# Autodesk Inventor assembly: BG_Mattenwagen
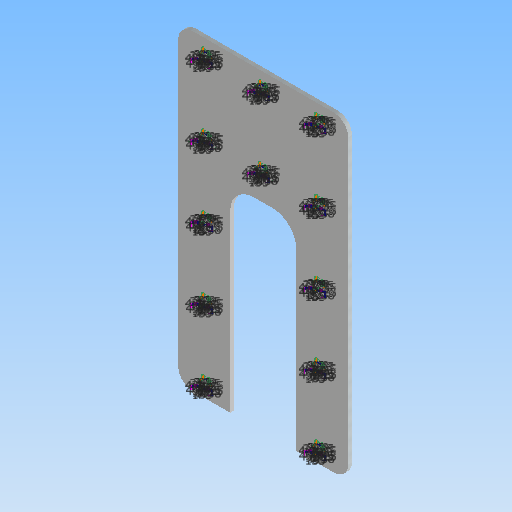
[picture p0: Inventor's stored thumbnail of the model, 512x512]
Saved by Autodesk Inventor 2024.4 (Build 284460000, 460)
## iProperties
Created: 2026-01-22
Part Number: BG_Mattenwagen
Document SubType Name: Assembly
Designer: windows-desktop
Mass: 56051.1 g
Surface Area: 201169 cm^2
Volume: 54823 cm^3
Density: 1.0224 g/cm^3
Author: windows-desktop
## Documents named in this file (4)
- C:\Users\windows-desktop\Desktop\Studium\Konstruktion\VaultWorkspace\Daten\I60-Konstruktion\I60-Gruppe-4\Bluhm\Daten\I60-Konstruktion\I60-Gruppe-4\Bluhm\Transport\BG_Mattenwagen.iam
- C:\Users\windows-desktop\Desktop\Studium\Konstruktion\VaultWorkspace\Daten\I60-Konstruktion\I60-Gruppe-4\Bluhm\Daten\I60-Konstruktion\I60-Gruppe-4\Bluhm\Transport\Wagen_Platte.ipt
- C:\Users\windows-desktop\Desktop\Studium\Konstruktion\VaultWorkspace\Daten\I60-Konstruktion\I60-Gruppe-4\Bluhm\Daten\I60-Konstruktion\I60-Gruppe-4\Bluhm\Transport\BG_Rolle.iam
- C:\Users\windows-desktop\Desktop\Studium\Konstruktion\VaultWorkspace\Daten\I60-Konstruktion\I60-Gruppe-4\Bluhm\Normteile\de-DE\ISO 4762(1)\DIN EN ISO 4762 - M10 x 16.ipt
## Components (61 placed, 3 different names)
1. Wagen_Platte:1 — Einfügen:1, Einfügen:2, Einfügen:3, Einfügen:4, Einfügen:5, Einfügen:6, Passend:1, Passend:3, Passend:5, Passend:7, Passend:9, Passend:11, Passend:13, Passend:15, Passend:17, Passend:19, Passend:21, Passend:23, Passend:25, Passend:27, Passend:29, Passend:31, Passend:33, Passend:35, Passend:37, Passend:39, Passend:41, Passend:43, Passend:45, Passend:47, Passend:49, Passend:51, Passend:53, Passend:55, Passend:57, Passend:59, Passend:61, Passend:63, Passend:65, Passend:67, Passend:69, Passend:71, Passend:73, Passend:75, Passend:77, Passend:79, Passend:81, Passend:83, Passend:85, Passend:87, Passend:89, Passend:91, Passend:93, Passend:95
2. DIN EN ISO 4762 M10 x 16:1 — Passend:1, Passend:2
3. DIN EN ISO 4762 M10 x 16:2 — Passend:3, Passend:4
4. DIN EN ISO 4762 M10 x 16:3 — Passend:5, Passend:6
5. DIN EN ISO 4762 M10 x 16:4 — Passend:7, Passend:8
6. DIN EN ISO 4762 M10 x 16:5 — Passend:9, Passend:10
7. DIN EN ISO 4762 M10 x 16:6 — Passend:11, Passend:12
8. DIN EN ISO 4762 M10 x 16:7 — Passend:13, Passend:14
9. DIN EN ISO 4762 M10 x 16:8 — Passend:15, Passend:16
10. DIN EN ISO 4762 M10 x 16:9 — Passend:17, Passend:18
11. DIN EN ISO 4762 M10 x 16:10 — Passend:19, Passend:20
12. DIN EN ISO 4762 M10 x 16:11 — Passend:21, Passend:22
13. DIN EN ISO 4762 M10 x 16:12 — Passend:23, Passend:24
14. DIN EN ISO 4762 M10 x 16:13 — Passend:25, Passend:26
15. DIN EN ISO 4762 M10 x 16:14 — Passend:27, Passend:28
16. DIN EN ISO 4762 M10 x 16:15 — Passend:29, Passend:30
17. DIN EN ISO 4762 M10 x 16:16 — Passend:31, Passend:32
18. DIN EN ISO 4762 M10 x 16:17 — Passend:33, Passend:34
19. DIN EN ISO 4762 M10 x 16:18 — Passend:35, Passend:36
20. DIN EN ISO 4762 M10 x 16:19 — Passend:37, Passend:38
21. DIN EN ISO 4762 M10 x 16:20 — Passend:39, Passend:40
22. DIN EN ISO 4762 M10 x 16:21 — Passend:41, Passend:42
23. DIN EN ISO 4762 M10 x 16:22 — Passend:43, Passend:44
24. DIN EN ISO 4762 M10 x 16:23 — Passend:45, Passend:46
25. DIN EN ISO 4762 M10 x 16:24 — Passend:47, Passend:48
26. DIN EN ISO 4762 M10 x 16:25 — Passend:49, Passend:50
27. DIN EN ISO 4762 M10 x 16:26 — Passend:51, Passend:52
28. DIN EN ISO 4762 M10 x 16:27 — Passend:53, Passend:54
29. DIN EN ISO 4762 M10 x 16:28 — Passend:55, Passend:56
30. DIN EN ISO 4762 M10 x 16:29 — Passend:57, Passend:58
31. DIN EN ISO 4762 M10 x 16:30 — Passend:59, Passend:60
32. DIN EN ISO 4762 M10 x 16:31 — Passend:61, Passend:62
33. DIN EN ISO 4762 M10 x 16:32 — Passend:63, Passend:64
34. DIN EN ISO 4762 M10 x 16:33 — Passend:65, Passend:66
35. DIN EN ISO 4762 M10 x 16:34 — Passend:67, Passend:68
36. DIN EN ISO 4762 M10 x 16:35 — Passend:69, Passend:70
37. DIN EN ISO 4762 M10 x 16:36 — Passend:71, Passend:72
38. DIN EN ISO 4762 M10 x 16:37 — Passend:73, Passend:74
39. DIN EN ISO 4762 M10 x 16:38 — Passend:75, Passend:76
40. DIN EN ISO 4762 M10 x 16:39 — Passend:77, Passend:78
41. DIN EN ISO 4762 M10 x 16:40 — Passend:79, Passend:80
42. DIN EN ISO 4762 M10 x 16:41 — Passend:81, Passend:82
43. DIN EN ISO 4762 M10 x 16:42 — Passend:83, Passend:84
44. DIN EN ISO 4762 M10 x 16:43 — Passend:85, Passend:86
45. DIN EN ISO 4762 M10 x 16:44 — Passend:87, Passend:88
46. DIN EN ISO 4762 M10 x 16:45 — Passend:89, Passend:90
47. DIN EN ISO 4762 M10 x 16:46 — Passend:91, Passend:92
48. DIN EN ISO 4762 M10 x 16:47 — Passend:93, Passend:94
49. DIN EN ISO 4762 M10 x 16:48 — Passend:95, Passend:96
50. BG_Rolle:3 [sub-assembly] — Einfügen:1, Einfügen:2
51. BG_Rolle:4 [sub-assembly]
52. BG_Rolle:5 [sub-assembly]
53. BG_Rolle:6 [sub-assembly]
54. BG_Rolle:7 [sub-assembly]
55. BG_Rolle:1 [sub-assembly] — Einfügen:3, Einfügen:4
56. BG_Rolle:8 [sub-assembly]
57. BG_Rolle:9 [sub-assembly] — Einfügen:5, Einfügen:6
58. BG_Rolle:10 [sub-assembly]
59. BG_Rolle:11 [sub-assembly]
60. BG_Rolle:12 [sub-assembly] — Passend:2, Passend:4, Passend:6, Passend:8, Passend:10, Passend:12, Passend:14, Passend:16, Passend:18, Passend:20, Passend:22, Passend:24, Passend:26, Passend:28, Passend:30, Passend:32, Passend:34, Passend:36, Passend:38, Passend:40, Passend:42, Passend:44, Passend:46, Passend:48, Passend:50, Passend:52, Passend:54, Passend:56, Passend:58, Passend:60, Passend:62, Passend:64, Passend:66, Passend:68, Passend:70, Passend:72, Passend:74, Passend:76, Passend:78, Passend:80, Passend:82, Passend:84, Passend:86, Passend:88, Passend:90, Passend:92, Passend:94, Passend:96
61. BG_Rolle:13 [sub-assembly]
## Component patterns: (5 elements, first: BG_Rolle:3), (2 elements, first: BG_Rolle:1), (5 elements, first: BG_Rolle:9)
## Relationships (102: Mate 96, Insert 6)
- Einfügen:1 [Insert]: Wagen_Platte:1 ↔ BG_Rolle:3
- Einfügen:2 [Insert]: Wagen_Platte:1 ↔ BG_Rolle:3
- Einfügen:3 [Insert]: Wagen_Platte:1 ↔ BG_Rolle:1
- Einfügen:4 [Insert]: Wagen_Platte:1 ↔ BG_Rolle:1
- Einfügen:5 [Insert]: Wagen_Platte:1 ↔ BG_Rolle:9
- Einfügen:6 [Insert]: Wagen_Platte:1 ↔ BG_Rolle:9
- Passend:1 [Mate]: Wagen_Platte:1 ↔ DIN EN ISO 4762 M10 x 16:1
- Passend:2 [Mate]: DIN EN ISO 4762 M10 x 16:1 ↔ BG_Rolle:12
- Passend:3 [Mate]: Wagen_Platte:1 ↔ DIN EN ISO 4762 M10 x 16:2
- Passend:4 [Mate]: DIN EN ISO 4762 M10 x 16:2 ↔ BG_Rolle:12
- Passend:5 [Mate]: Wagen_Platte:1 ↔ DIN EN ISO 4762 M10 x 16:3
- Passend:6 [Mate]: DIN EN ISO 4762 M10 x 16:3 ↔ BG_Rolle:12
- Passend:7 [Mate]: Wagen_Platte:1 ↔ DIN EN ISO 4762 M10 x 16:4
- Passend:8 [Mate]: DIN EN ISO 4762 M10 x 16:4 ↔ BG_Rolle:12
- Passend:9 [Mate]: Wagen_Platte:1 ↔ DIN EN ISO 4762 M10 x 16:5
- Passend:10 [Mate]: DIN EN ISO 4762 M10 x 16:5 ↔ BG_Rolle:12
- Passend:11 [Mate]: Wagen_Platte:1 ↔ DIN EN ISO 4762 M10 x 16:6
- Passend:12 [Mate]: DIN EN ISO 4762 M10 x 16:6 ↔ BG_Rolle:12
- Passend:13 [Mate]: Wagen_Platte:1 ↔ DIN EN ISO 4762 M10 x 16:7
- Passend:14 [Mate]: DIN EN ISO 4762 M10 x 16:7 ↔ BG_Rolle:12
- Passend:15 [Mate]: Wagen_Platte:1 ↔ DIN EN ISO 4762 M10 x 16:8
- Passend:16 [Mate]: DIN EN ISO 4762 M10 x 16:8 ↔ BG_Rolle:12
- Passend:17 [Mate]: Wagen_Platte:1 ↔ DIN EN ISO 4762 M10 x 16:9
- Passend:18 [Mate]: DIN EN ISO 4762 M10 x 16:9 ↔ BG_Rolle:12
- Passend:19 [Mate]: Wagen_Platte:1 ↔ DIN EN ISO 4762 M10 x 16:10
- Passend:20 [Mate]: DIN EN ISO 4762 M10 x 16:10 ↔ BG_Rolle:12
- Passend:21 [Mate]: Wagen_Platte:1 ↔ DIN EN ISO 4762 M10 x 16:11
- Passend:22 [Mate]: DIN EN ISO 4762 M10 x 16:11 ↔ BG_Rolle:12
- Passend:23 [Mate]: Wagen_Platte:1 ↔ DIN EN ISO 4762 M10 x 16:12
- Passend:24 [Mate]: DIN EN ISO 4762 M10 x 16:12 ↔ BG_Rolle:12
- Passend:25 [Mate]: Wagen_Platte:1 ↔ DIN EN ISO 4762 M10 x 16:13
- Passend:26 [Mate]: DIN EN ISO 4762 M10 x 16:13 ↔ BG_Rolle:12
- Passend:27 [Mate]: Wagen_Platte:1 ↔ DIN EN ISO 4762 M10 x 16:14
- Passend:28 [Mate]: DIN EN ISO 4762 M10 x 16:14 ↔ BG_Rolle:12
- Passend:29 [Mate]: Wagen_Platte:1 ↔ DIN EN ISO 4762 M10 x 16:15
- Passend:30 [Mate]: DIN EN ISO 4762 M10 x 16:15 ↔ BG_Rolle:12
- Passend:31 [Mate]: Wagen_Platte:1 ↔ DIN EN ISO 4762 M10 x 16:16
- Passend:32 [Mate]: DIN EN ISO 4762 M10 x 16:16 ↔ BG_Rolle:12
- Passend:33 [Mate]: Wagen_Platte:1 ↔ DIN EN ISO 4762 M10 x 16:17
- Passend:34 [Mate]: DIN EN ISO 4762 M10 x 16:17 ↔ BG_Rolle:12
- Passend:35 [Mate]: Wagen_Platte:1 ↔ DIN EN ISO 4762 M10 x 16:18
- Passend:36 [Mate]: DIN EN ISO 4762 M10 x 16:18 ↔ BG_Rolle:12
- Passend:37 [Mate]: Wagen_Platte:1 ↔ DIN EN ISO 4762 M10 x 16:19
- Passend:38 [Mate]: DIN EN ISO 4762 M10 x 16:19 ↔ BG_Rolle:12
- Passend:39 [Mate]: Wagen_Platte:1 ↔ DIN EN ISO 4762 M10 x 16:20
- Passend:40 [Mate]: DIN EN ISO 4762 M10 x 16:20 ↔ BG_Rolle:12
- Passend:41 [Mate]: Wagen_Platte:1 ↔ DIN EN ISO 4762 M10 x 16:21
- Passend:42 [Mate]: DIN EN ISO 4762 M10 x 16:21 ↔ BG_Rolle:12
- Passend:43 [Mate]: Wagen_Platte:1 ↔ DIN EN ISO 4762 M10 x 16:22
- Passend:44 [Mate]: DIN EN ISO 4762 M10 x 16:22 ↔ BG_Rolle:12
- Passend:45 [Mate]: Wagen_Platte:1 ↔ DIN EN ISO 4762 M10 x 16:23
- Passend:46 [Mate]: DIN EN ISO 4762 M10 x 16:23 ↔ BG_Rolle:12
- Passend:47 [Mate]: Wagen_Platte:1 ↔ DIN EN ISO 4762 M10 x 16:24
- Passend:48 [Mate]: DIN EN ISO 4762 M10 x 16:24 ↔ BG_Rolle:12
- Passend:49 [Mate]: Wagen_Platte:1 ↔ DIN EN ISO 4762 M10 x 16:25
- Passend:50 [Mate]: DIN EN ISO 4762 M10 x 16:25 ↔ BG_Rolle:12
- Passend:51 [Mate]: Wagen_Platte:1 ↔ DIN EN ISO 4762 M10 x 16:26
- Passend:52 [Mate]: DIN EN ISO 4762 M10 x 16:26 ↔ BG_Rolle:12
- Passend:53 [Mate]: Wagen_Platte:1 ↔ DIN EN ISO 4762 M10 x 16:27
- Passend:54 [Mate]: DIN EN ISO 4762 M10 x 16:27 ↔ BG_Rolle:12
- Passend:55 [Mate]: Wagen_Platte:1 ↔ DIN EN ISO 4762 M10 x 16:28
- Passend:56 [Mate]: DIN EN ISO 4762 M10 x 16:28 ↔ BG_Rolle:12
- Passend:57 [Mate]: Wagen_Platte:1 ↔ DIN EN ISO 4762 M10 x 16:29
- Passend:58 [Mate]: DIN EN ISO 4762 M10 x 16:29 ↔ BG_Rolle:12
- Passend:59 [Mate]: Wagen_Platte:1 ↔ DIN EN ISO 4762 M10 x 16:30
- Passend:60 [Mate]: DIN EN ISO 4762 M10 x 16:30 ↔ BG_Rolle:12
- Passend:61 [Mate]: Wagen_Platte:1 ↔ DIN EN ISO 4762 M10 x 16:31
- Passend:62 [Mate]: DIN EN ISO 4762 M10 x 16:31 ↔ BG_Rolle:12
- Passend:63 [Mate]: Wagen_Platte:1 ↔ DIN EN ISO 4762 M10 x 16:32
- Passend:64 [Mate]: DIN EN ISO 4762 M10 x 16:32 ↔ BG_Rolle:12
- Passend:65 [Mate]: Wagen_Platte:1 ↔ DIN EN ISO 4762 M10 x 16:33
- Passend:66 [Mate]: DIN EN ISO 4762 M10 x 16:33 ↔ BG_Rolle:12
- Passend:67 [Mate]: Wagen_Platte:1 ↔ DIN EN ISO 4762 M10 x 16:34
- Passend:68 [Mate]: DIN EN ISO 4762 M10 x 16:34 ↔ BG_Rolle:12
- Passend:69 [Mate]: Wagen_Platte:1 ↔ DIN EN ISO 4762 M10 x 16:35
- Passend:70 [Mate]: DIN EN ISO 4762 M10 x 16:35 ↔ BG_Rolle:12
- Passend:71 [Mate]: Wagen_Platte:1 ↔ DIN EN ISO 4762 M10 x 16:36
- Passend:72 [Mate]: DIN EN ISO 4762 M10 x 16:36 ↔ BG_Rolle:12
- Passend:73 [Mate]: Wagen_Platte:1 ↔ DIN EN ISO 4762 M10 x 16:37
- Passend:74 [Mate]: DIN EN ISO 4762 M10 x 16:37 ↔ BG_Rolle:12
- Passend:75 [Mate]: Wagen_Platte:1 ↔ DIN EN ISO 4762 M10 x 16:38
- Passend:76 [Mate]: DIN EN ISO 4762 M10 x 16:38 ↔ BG_Rolle:12
- Passend:77 [Mate]: Wagen_Platte:1 ↔ DIN EN ISO 4762 M10 x 16:39
- Passend:78 [Mate]: DIN EN ISO 4762 M10 x 16:39 ↔ BG_Rolle:12
- Passend:79 [Mate]: Wagen_Platte:1 ↔ DIN EN ISO 4762 M10 x 16:40
- Passend:80 [Mate]: DIN EN ISO 4762 M10 x 16:40 ↔ BG_Rolle:12
- Passend:81 [Mate]: Wagen_Platte:1 ↔ DIN EN ISO 4762 M10 x 16:41
- Passend:82 [Mate]: DIN EN ISO 4762 M10 x 16:41 ↔ BG_Rolle:12
- Passend:83 [Mate]: Wagen_Platte:1 ↔ DIN EN ISO 4762 M10 x 16:42
- Passend:84 [Mate]: DIN EN ISO 4762 M10 x 16:42 ↔ BG_Rolle:12
- Passend:85 [Mate]: Wagen_Platte:1 ↔ DIN EN ISO 4762 M10 x 16:43
- Passend:86 [Mate]: DIN EN ISO 4762 M10 x 16:43 ↔ BG_Rolle:12
- Passend:87 [Mate]: Wagen_Platte:1 ↔ DIN EN ISO 4762 M10 x 16:44
- Passend:88 [Mate]: DIN EN ISO 4762 M10 x 16:44 ↔ BG_Rolle:12
- Passend:89 [Mate]: Wagen_Platte:1 ↔ DIN EN ISO 4762 M10 x 16:45
- Passend:90 [Mate]: DIN EN ISO 4762 M10 x 16:45 ↔ BG_Rolle:12
- Passend:91 [Mate]: Wagen_Platte:1 ↔ DIN EN ISO 4762 M10 x 16:46
- Passend:92 [Mate]: DIN EN ISO 4762 M10 x 16:46 ↔ BG_Rolle:12
- Passend:93 [Mate]: Wagen_Platte:1 ↔ DIN EN ISO 4762 M10 x 16:47
- Passend:94 [Mate]: DIN EN ISO 4762 M10 x 16:47 ↔ BG_Rolle:12
- Passend:95 [Mate]: Wagen_Platte:1 ↔ DIN EN ISO 4762 M10 x 16:48
- Passend:96 [Mate]: DIN EN ISO 4762 M10 x 16:48 ↔ BG_Rolle:12
